# Autodesk Inventor assembly: fc17-120
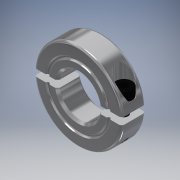
[picture p0: Inventor's stored thumbnail of the model, 180x180]
Saved by Autodesk Inventor 2017.1 (Build 211199000, 199)
## iProperties
Category: Miscellaneous
Company: Autodesk Inc.
Created: 2016-12-20
Part Number: fc17-120
Document SubType Name: Assembly
Designer: Autodesk Inc.
Catalog Web Link: http://www.ruland.com/shaft-collar.php?recordID=ENSP20-6-A
Vendor: Ruland
Author: Autodesk Inc.
Keywords: FIRST Choice
## Documents named in this file (3)
- D:\FIRST\FIRST KOP 2017\FIRST FirstChoice 2017\fc17-120_ShaftCollar.iam
- D:\FIRST\FIRST KOP 2017\FIRST FirstChoice 2017\Parts\MISC_Collar_ENSP20-6-A.ipt
- D:\FIRST\FIRST KOP 2017\FIRST FirstChoice 2017\Parts\ISO 4762 - M2 x 6ISO.ipt
## Components (3 placed, 2 different names)
1. MISC_Collar_ENSP20-6-A:1 — Insert:1, Insert:2
2. ISO 4762 M2 x 6:1 — Insert:1
3. ISO 4762 M2 x 6:2 — Insert:2
## Relationships (2: Insert 2)
- Insert:1: MISC_Collar_ENSP20-6-A:1 ↔ ISO 4762 M2 x 6:1
- Insert:2: MISC_Collar_ENSP20-6-A:1 ↔ ISO 4762 M2 x 6:2
